# Autodesk Inventor assembly: 100mm omuniwheel_MIR_MIR
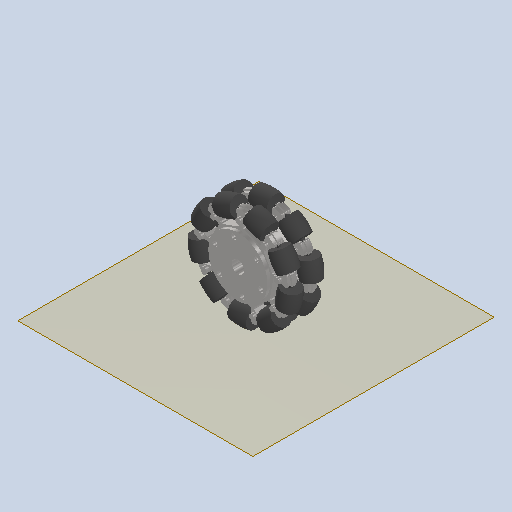
[picture p0: Inventor's stored thumbnail of the model, 512x512]
Saved by Autodesk Inventor 2025.1 (Build 291241000, 241)
## iProperties
Created: 2023-11-21
Part Number: 100mm omuniwheel_MIR_MIR
Document SubType Name: Assembly
Designer: haruy
Author: fhbdh
## Documents named in this file (6)
- C:\Users\haruy\Documents\ロボコン\NHK2025\cad\nagahisa\base_weel\takagi_weel\Workspaces\作業スペース\takagi\omuni_wheel_ver3.0\parts\frequently used parts\タイヤ\omni wheel\100mm wheel\100mm omuniwheel_MIR_MIR.iam
- C:\Users\haruy\Documents\ロボコン\NHK2025\cad\nagahisa\base_weel\takagi_weel\Workspaces\作業スペース\takagi\omuni_wheel_ver2.0\parts\frequently used parts\タイヤ\omni wheel\100mm wheel\omuni_flame_MIR_MIR.ipt
- C:\Users\haruy\Documents\ロボコン\NHK2025\cad\nagahisa\base_weel\takagi_weel\Workspaces\作業スペース\takagi\omuni_wheel_ver2.0\parts\frequently used parts\タイヤ\omni wheel\100mm wheel\omuni_rubber_MIR_MIR.ipt
- C:\Users\haruy\Documents\ロボコン\NHK2025\cad\nagahisa\base_weel\takagi_weel\Workspaces\作業スペース\takagi\omuni_wheel_ver2.0\parts\frequently used parts\タイヤ\omni wheel\100mm wheel\frange_MIR_MIR.ipt
- C:\Users\haruy\Documents\ロボコン\NHK2025\cad\nagahisa\base_weel\takagi_weel\Workspaces\作業スペース\takagi\omuni_wheel_ver2.0\parts\frequently used parts\タイヤ\omni wheel\100mm wheel\al_shaft_MIR_MIR.ipt
- C:\Users\haruy\Documents\ロボコン\NHK2025\cad\nagahisa\base_weel\takagi_weel\Workspaces\作業スペース\takagi\omuni_wheel_ver2.0\parts\frequently used parts\タイヤ\omni wheel\100mm wheel\nut_MIR_MIR.ipt
## Components (27 placed, 5 different names)
1. omuni_flame_MIR_MIR:1 — 挿入:3, 挿入:4, 挿入:5, 挿入:9, 挿入:8, 挿入:7, 挿入:2, 挿入:6, 挿入:1, 挿入:19, メイト:1, 挿入:22, 挿入:21, 挿入:20
2. omuni_rubber_MIR_MIR:1 — 挿入:3
3. omuni_rubber_MIR_MIR:2 — 挿入:4
4. omuni_rubber_MIR_MIR:3 — 挿入:5
5. omuni_rubber_MIR_MIR:4 — 挿入:9
6. omuni_rubber_MIR_MIR:5 — 挿入:8
7. omuni_rubber_MIR_MIR:6 — 挿入:7
8. omuni_rubber_MIR_MIR:7 — 挿入:2
9. omuni_rubber_MIR_MIR:8 — 挿入:6
10. omuni_rubber_MIR_MIR:9 — 挿入:1, メイト:3
11. frange_MIR_MIR:1 — 挿入:19, メイト:1
12. omuni_flame_MIR_MIR:2 — メイト:2, 挿入:12, 挿入:13, 挿入:14, 挿入:18, 挿入:17, 挿入:16, 挿入:11, 挿入:15, 挿入:10, 挿入:28, 挿入:29, 挿入:32, 挿入:30, 挿入:31
13. omuni_rubber_MIR_MIR:10 — 挿入:12
14. omuni_rubber_MIR_MIR:11 — 挿入:13
15. omuni_rubber_MIR_MIR:12 — 挿入:14
16. omuni_rubber_MIR_MIR:13 — 挿入:18
17. omuni_rubber_MIR_MIR:14 — 挿入:17
18. omuni_rubber_MIR_MIR:15 — 挿入:16
19. omuni_rubber_MIR_MIR:16 — 挿入:11
20. omuni_rubber_MIR_MIR:17 — 挿入:15
21. omuni_rubber_MIR_MIR:18 — 挿入:10, 正接:1
22. al_shaft_MIR_MIR:1 — 挿入:22, 挿入:28
23. al_shaft_MIR_MIR:2 — 挿入:21, 挿入:29
24. al_shaft_MIR_MIR:3 — 挿入:20
25. nut_MIR_MIR:1 — 挿入:32
26. nut_MIR_MIR:2 — 挿入:30
27. nut_MIR_MIR:3 — 挿入:31
## Relationships (31: Insert 27, Mate 3, Tangent 1)
- 挿入:3 [Insert]: omuni_flame_MIR_MIR:1 ↔ omuni_rubber_MIR_MIR:1
- 挿入:4 [Insert]: omuni_flame_MIR_MIR:1 ↔ omuni_rubber_MIR_MIR:2
- 挿入:5 [Insert]: omuni_flame_MIR_MIR:1 ↔ omuni_rubber_MIR_MIR:3
- 挿入:9 [Insert]: omuni_flame_MIR_MIR:1 ↔ omuni_rubber_MIR_MIR:4
- 挿入:8 [Insert]: omuni_flame_MIR_MIR:1 ↔ omuni_rubber_MIR_MIR:5
- 挿入:7 [Insert]: omuni_flame_MIR_MIR:1 ↔ omuni_rubber_MIR_MIR:6
- 挿入:2 [Insert]: omuni_flame_MIR_MIR:1 ↔ omuni_rubber_MIR_MIR:7
- 挿入:6 [Insert]: omuni_flame_MIR_MIR:1 ↔ omuni_rubber_MIR_MIR:8
- 挿入:1 [Insert]: omuni_flame_MIR_MIR:1 ↔ omuni_rubber_MIR_MIR:9
- メイト:3 [Mate]: omuni_rubber_MIR_MIR:9
- 挿入:19 [Insert]: omuni_flame_MIR_MIR:1 ↔ frange_MIR_MIR:1
- メイト:1 [Mate]: omuni_flame_MIR_MIR:1 ↔ frange_MIR_MIR:1
- メイト:2 [Mate]: omuni_flame_MIR_MIR:2
- 挿入:12 [Insert]: omuni_flame_MIR_MIR:2 ↔ omuni_rubber_MIR_MIR:10
- 挿入:13 [Insert]: omuni_flame_MIR_MIR:2 ↔ omuni_rubber_MIR_MIR:11
- 挿入:14 [Insert]: omuni_flame_MIR_MIR:2 ↔ omuni_rubber_MIR_MIR:12
- 挿入:18 [Insert]: omuni_flame_MIR_MIR:2 ↔ omuni_rubber_MIR_MIR:13
- 挿入:17 [Insert]: omuni_flame_MIR_MIR:2 ↔ omuni_rubber_MIR_MIR:14
- 挿入:16 [Insert]: omuni_flame_MIR_MIR:2 ↔ omuni_rubber_MIR_MIR:15
- 挿入:11 [Insert]: omuni_flame_MIR_MIR:2 ↔ omuni_rubber_MIR_MIR:16
- 挿入:15 [Insert]: omuni_flame_MIR_MIR:2 ↔ omuni_rubber_MIR_MIR:17
- 挿入:10 [Insert]: omuni_flame_MIR_MIR:2 ↔ omuni_rubber_MIR_MIR:18
- 正接:1 [Tangent]: omuni_rubber_MIR_MIR:18
- 挿入:22 [Insert]: omuni_flame_MIR_MIR:1 ↔ al_shaft_MIR_MIR:1
- 挿入:28 [Insert]: omuni_flame_MIR_MIR:2 ↔ al_shaft_MIR_MIR:1
- 挿入:21 [Insert]: omuni_flame_MIR_MIR:1 ↔ al_shaft_MIR_MIR:2
- 挿入:29 [Insert]: omuni_flame_MIR_MIR:2 ↔ al_shaft_MIR_MIR:2
- 挿入:20 [Insert]: omuni_flame_MIR_MIR:1 ↔ al_shaft_MIR_MIR:3
- 挿入:32 [Insert]: omuni_flame_MIR_MIR:2 ↔ nut_MIR_MIR:1
- 挿入:30 [Insert]: omuni_flame_MIR_MIR:2 ↔ nut_MIR_MIR:2
- 挿入:31 [Insert]: omuni_flame_MIR_MIR:2 ↔ nut_MIR_MIR:3
